# Autodesk Inventor assembly: Rigid Coupling 5,8
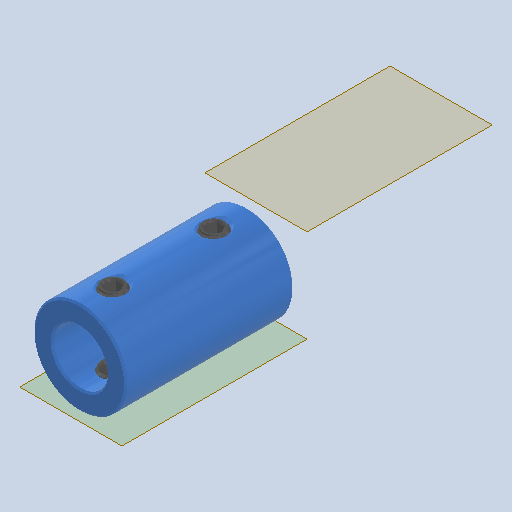
[picture p0: Inventor's stored thumbnail of the model, 512x512]
Saved by Autodesk Inventor 2025.2 (Build 292293000, 293)
## iProperties
Created: 2025-05-30
Part Number: Rigid Coupling 5,8
Document SubType Name: Assembly
Designer: Simon
Author: Simon
## Documents named in this file (3)
- C:\Users\Simon\OneDrive\Documents\Inventor\Skripsie2025\PartsFolder\Rigid Coupling 5,8\Rigid Coupling 5,8.iam
- C:\Users\Simon\OneDrive\Documents\Inventor\Skripsie2025\PartsFolder\Rigid Coupling 5,8\Rigid Coupler 5,8.ipt
- C:\Users\Simon\OneDrive\Documents\Inventor\Skripsie2025\PartsFolder\Rigid Coupling 5,8\M4 Screw.ipt
## Components (5 placed, 2 different names)
1. Rigid Coupler 5,8:1 — Mate:1, Mate:2, Mate:3, Mate:4, Tangent:1, Tangent:2
2. M4 Screw:1 — Mate:2, Flush:2
3. M4 Screw:2 — Mate:4, Flush:1, Angle:2
4. M4 Screw:3 — Mate:1, Flush:2, Angle:1, Flush:3
5. M4 Screw:4 — Mate:3, Flush:1, Flush:4
## Relationships (12: Mate 4, Flush 4, Angle 2, Tangent 2)
- Mate:1: Rigid Coupler 5,8:1 ↔ M4 Screw:3
- Mate:2: Rigid Coupler 5,8:1 ↔ M4 Screw:1
- Mate:3: Rigid Coupler 5,8:1 ↔ M4 Screw:4
- Mate:4: Rigid Coupler 5,8:1 ↔ M4 Screw:2
- Flush:1: M4 Screw:2 ↔ M4 Screw:4
- Flush:2: M4 Screw:1 ↔ M4 Screw:3
- Angle:1 (0 deg): M4 Screw:3
- Tangent:1: Rigid Coupler 5,8:1
- Angle:2 (0 deg): M4 Screw:2
- Tangent:2: Rigid Coupler 5,8:1
- Flush:3: M4 Screw:3
- Flush:4: M4 Screw:4
